# Autodesk Inventor assembly: XY Joint-Unit [A]
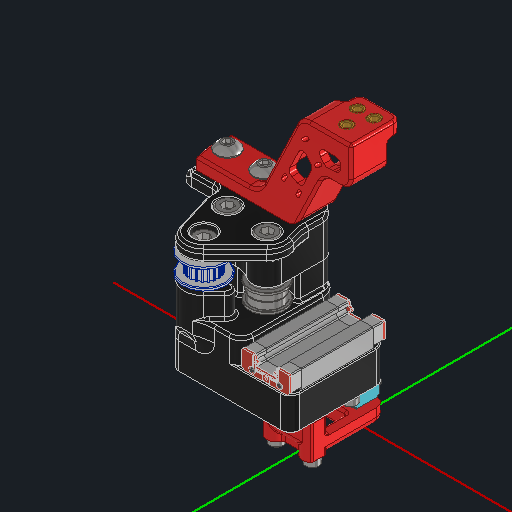
[picture p0: Inventor's stored thumbnail of the model, 512x512]
Saved by Autodesk Inventor 2022.2 (Build 262287010, 287A)
## iProperties
Created: 2022-03-15
Part Number: XY Joint-Unit [A]
Document SubType Name: Assembly
Designer: sleib
Author: sleib
## Documents named in this file (16)
- C:\Users\sleib\Projekte\Voron-2\CAD\Inventor\XY Joint-Unit [A].iam
- C:\Users\sleib\Projekte\Voron-2\CAD\Inventor\MGN9H Carriage.ipt
- C:\Users\sleib\Projekte\Voron-2\CAD\Inventor\M3x16 SHCS.ipt
- C:\Users\sleib\Projekte\Voron-2\CAD\Inventor\M3x30 SHCS.ipt
- C:\Users\sleib\Projekte\Voron-2\CAD\Inventor\M5x40 SHCS.ipt
- C:\Users\sleib\Projekte\Voron-2\CAD\Inventor\GT2 20T Idler (6mm).ipt
- C:\Users\sleib\Projekte\Voron-2\CAD\Inventor\M5 Hexnut.ipt
- C:\Users\sleib\Projekte\Voron-2\CAD\Inventor\M5 Spacer (1mm).ipt
- C:\Users\sleib\Projekte\Voron-2\CAD\Inventor\Bearing F695-ZZ.ipt
- C:\Users\sleib\Projekte\Voron-2\CAD\Inventor\Chain Standoff (3-Hole).ipt
- C:\Users\sleib\Projekte\Voron-2\CAD\Inventor\M5x16 BHCS.ipt
- C:\Users\sleib\Projekte\Voron-2\CAD\Inventor\M5x30 BHCS.ipt
- C:\Users\sleib\Projekte\Voron-2\CAD\Inventor\XY Joint MGN12H [A].ipt
- C:\Users\sleib\Projekte\Voron-2\CAD\Inventor\M3 Threaded Insert.ipt
- C:\Users\sleib\Projekte\Voron-2\CAD\Inventor\Y Endstop Mount (Panasonic).ipt
- C:\Users\sleib\Projekte\Voron-2\CAD\Inventor\Microswitch Panasonic.ipt
## Components (28 placed, 15 different names)
1. XY Joint MGN12H [A]:1 — Passend:50, Passend:51, Passend:52, Passend:53, Passend:54, Passend:55, Passend:56, Passend:57, Winkel:1, Winkel:2, Winkel:3, Passend:58, Passend:59, Passend:60, Passend:61, Passend:62, Passend:63, Passend:64, Passend:65, Passend:66, Passend:67, Passend:69, Passend:70, Passend:71, Passend:72, Passend:73, Passend:75, Passend:76, Passend:78, Passend:80, Passend:81, Passend:83, Passend:84, Passend:96
2. MGN9H Carriage:1 — Passend:10, Passend:11, Passend:12, Passend:13, Passend:69
3. GT2 20T Idler (6mm):1 — Passend:23, Passend:83
4. Bearing F695-ZZ:1 — Passend:37, Passend:40, Passend:41
5. Bearing F695-ZZ:2 — Passend:38, Passend:41, Passend:42
6. M3x16 SHCS:1 — Passend:10, Passend:65, Passend:71
7. M3x16 SHCS:2 — Passend:11, Passend:64, Passend:70
8. M3x30 SHCS:1 — Passend:12, Passend:67, Passend:92, Passend:94
9. M3x30 SHCS:2 — Passend:13, Passend:66, Passend:93, Passend:95
10. M5x40 SHCS:1 — Passend:23, Passend:81, Passend:84
11. M5x40 SHCS:2 — Passend:36, Passend:37, Passend:38, Passend:39, Passend:74, Passend:76
12. M5x40 SHCS:3 — Passend:79, Passend:80
13. M5x40 SHCS:4 — Passend:77, Passend:78
14. M5 Hexnut:1 — Passend:50, Winkel:2, Passend:60, Passend:79
15. M5 Hexnut:2 — Passend:51, Winkel:1, Passend:58, Passend:74
16. M5 Hexnut:3 — Passend:52, Winkel:3, Passend:59, Passend:77
17. M5 Spacer (1mm):1 — Passend:36, Passend:40
18. M5 Spacer (1mm):2 — Passend:39, Passend:42, Passend:75
19. Chain Standoff (3-Hole):1 — Passend:46, Passend:47, Passend:48, Passend:49, Passend:63, Passend:85, Passend:86, Passend:87, Fluchtend:1, Fluchtend:2, Fluchtend:3
20. M5x16 BHCS:1 — Passend:46, Passend:48, Passend:61
21. M5x16 BHCS:2 — Passend:47, Passend:49, Passend:62
22. M5x30 BHCS:1 — Passend:72, Passend:73
23. M3 Threaded Insert:1 — Passend:86, Fluchtend:1
24. M3 Threaded Insert:2 — Passend:87, Fluchtend:2
25. M3 Threaded Insert:3 — Passend:85, Fluchtend:3
26. Y Endstop Mount (Panasonic):1 — Passend:88, Fluchtend:4, Passend:89, Passend:91, Passend:92, Passend:93, Passend:94, Passend:95, Passend:96
27. M3 Threaded Insert:4 — Passend:88, Fluchtend:4, Passend:90
28. Microswitch Panasonic:1 — Passend:89, Passend:90, Passend:91
## Relationships (68: Mate 61, Flush 4, Angle 3)
- Passend:10 [Mate]: MGN9H Carriage:1 ↔ M3x16 SHCS:1
- Passend:11 [Mate]: MGN9H Carriage:1 ↔ M3x16 SHCS:2
- Passend:12 [Mate]: MGN9H Carriage:1 ↔ M3x30 SHCS:1
- Passend:13 [Mate]: MGN9H Carriage:1 ↔ M3x30 SHCS:2
- Passend:23 [Mate]: GT2 20T Idler (6mm):1 ↔ M5x40 SHCS:1
- Passend:36 [Mate]: M5x40 SHCS:2 ↔ M5 Spacer (1mm):1
- Passend:37 [Mate]: Bearing F695-ZZ:1 ↔ M5x40 SHCS:2
- Passend:38 [Mate]: Bearing F695-ZZ:2 ↔ M5x40 SHCS:2
- Passend:39 [Mate]: M5x40 SHCS:2 ↔ M5 Spacer (1mm):2
- Passend:40 [Mate]: Bearing F695-ZZ:1 ↔ M5 Spacer (1mm):1
- Passend:41 [Mate]: Bearing F695-ZZ:1 ↔ Bearing F695-ZZ:2
- Passend:42 [Mate]: Bearing F695-ZZ:2 ↔ M5 Spacer (1mm):2
- Passend:46 [Mate]: Chain Standoff (3-Hole):1 ↔ M5x16 BHCS:1
- Passend:47 [Mate]: Chain Standoff (3-Hole):1 ↔ M5x16 BHCS:2
- Passend:48 [Mate]: Chain Standoff (3-Hole):1 ↔ M5x16 BHCS:1
- Passend:49 [Mate]: Chain Standoff (3-Hole):1 ↔ M5x16 BHCS:2
- Passend:50 [Mate]: XY Joint MGN12H [A]:1 ↔ M5 Hexnut:1
- Passend:51 [Mate]: XY Joint MGN12H [A]:1 ↔ M5 Hexnut:2
- Passend:52 [Mate]: XY Joint MGN12H [A]:1 ↔ M5 Hexnut:3
- Passend:53 [Mate]: XY Joint MGN12H [A]:1
- Passend:54 [Mate]: XY Joint MGN12H [A]:1
- Passend:55 [Mate]: XY Joint MGN12H [A]:1
- Passend:56 [Mate] (7.5 mm): XY Joint MGN12H [A]:1
- Passend:57 [Mate] (7.5 mm): XY Joint MGN12H [A]:1
- Winkel:1 [Angle] (0 deg): XY Joint MGN12H [A]:1 ↔ M5 Hexnut:2
- Winkel:2 [Angle] (0 deg): XY Joint MGN12H [A]:1 ↔ M5 Hexnut:1
- Winkel:3 [Angle] (0 deg): XY Joint MGN12H [A]:1 ↔ M5 Hexnut:3
- Passend:58 [Mate]: XY Joint MGN12H [A]:1 ↔ M5 Hexnut:2
- Passend:59 [Mate]: XY Joint MGN12H [A]:1 ↔ M5 Hexnut:3
- Passend:60 [Mate]: XY Joint MGN12H [A]:1 ↔ M5 Hexnut:1
- Passend:61 [Mate]: XY Joint MGN12H [A]:1 ↔ M5x16 BHCS:1
- Passend:62 [Mate]: XY Joint MGN12H [A]:1 ↔ M5x16 BHCS:2
- Passend:63 [Mate]: XY Joint MGN12H [A]:1 ↔ Chain Standoff (3-Hole):1
- Passend:64 [Mate]: XY Joint MGN12H [A]:1 ↔ M3x16 SHCS:2
- Passend:65 [Mate]: XY Joint MGN12H [A]:1 ↔ M3x16 SHCS:1
- Passend:66 [Mate]: XY Joint MGN12H [A]:1 ↔ M3x30 SHCS:2
- Passend:67 [Mate]: XY Joint MGN12H [A]:1 ↔ M3x30 SHCS:1
- Passend:69 [Mate]: XY Joint MGN12H [A]:1 ↔ MGN9H Carriage:1
- Passend:70 [Mate]: XY Joint MGN12H [A]:1 ↔ M3x16 SHCS:2
- Passend:71 [Mate]: XY Joint MGN12H [A]:1 ↔ M3x16 SHCS:1
- Passend:72 [Mate]: XY Joint MGN12H [A]:1 ↔ M5x30 BHCS:1
- Passend:73 [Mate]: XY Joint MGN12H [A]:1 ↔ M5x30 BHCS:1
- Passend:74 [Mate]: M5x40 SHCS:2 ↔ M5 Hexnut:2
- Passend:75 [Mate]: XY Joint MGN12H [A]:1 ↔ M5 Spacer (1mm):2
- Passend:76 [Mate]: XY Joint MGN12H [A]:1 ↔ M5x40 SHCS:2
- Passend:77 [Mate]: M5x40 SHCS:4 ↔ M5 Hexnut:3
- Passend:78 [Mate]: XY Joint MGN12H [A]:1 ↔ M5x40 SHCS:4
- Passend:79 [Mate]: M5x40 SHCS:3 ↔ M5 Hexnut:1
- Passend:80 [Mate]: XY Joint MGN12H [A]:1 ↔ M5x40 SHCS:3
- Passend:81 [Mate]: XY Joint MGN12H [A]:1 ↔ M5x40 SHCS:1
- Passend:83 [Mate]: XY Joint MGN12H [A]:1 ↔ GT2 20T Idler (6mm):1
- Passend:84 [Mate]: XY Joint MGN12H [A]:1 ↔ M5x40 SHCS:1
- Passend:85 [Mate]: Chain Standoff (3-Hole):1 ↔ M3 Threaded Insert:3
- Passend:86 [Mate]: Chain Standoff (3-Hole):1 ↔ M3 Threaded Insert:1
- Passend:87 [Mate]: Chain Standoff (3-Hole):1 ↔ M3 Threaded Insert:2
- Fluchtend:1 [Flush]: Chain Standoff (3-Hole):1 ↔ M3 Threaded Insert:1
- Fluchtend:2 [Flush]: Chain Standoff (3-Hole):1 ↔ M3 Threaded Insert:2
- Fluchtend:3 [Flush]: Chain Standoff (3-Hole):1 ↔ M3 Threaded Insert:3
- Passend:88 [Mate]: Y Endstop Mount (Panasonic):1 ↔ M3 Threaded Insert:4
- Fluchtend:4 [Flush]: Y Endstop Mount (Panasonic):1 ↔ M3 Threaded Insert:4
- Passend:89 [Mate]: Y Endstop Mount (Panasonic):1 ↔ Microswitch Panasonic:1
- Passend:90 [Mate]: M3 Threaded Insert:4 ↔ Microswitch Panasonic:1
- Passend:91 [Mate]: Y Endstop Mount (Panasonic):1 ↔ Microswitch Panasonic:1
- Passend:92 [Mate]: M3x30 SHCS:1 ↔ Y Endstop Mount (Panasonic):1
- Passend:93 [Mate]: M3x30 SHCS:2 ↔ Y Endstop Mount (Panasonic):1
- Passend:94 [Mate]: M3x30 SHCS:1 ↔ Y Endstop Mount (Panasonic):1
- Passend:95 [Mate]: M3x30 SHCS:2 ↔ Y Endstop Mount (Panasonic):1
- Passend:96 [Mate]: XY Joint MGN12H [A]:1 ↔ Y Endstop Mount (Panasonic):1
